# Autodesk Inventor assembly: RFO-Mounted
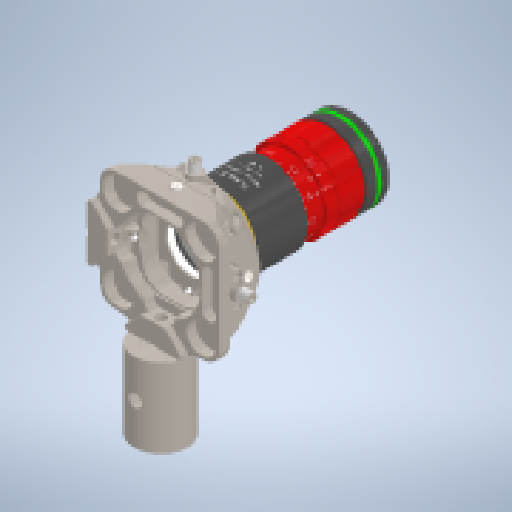
[picture p0: Inventor's stored thumbnail of the model, 512x512]
Saved by Autodesk Inventor 2024.2 (Build 282272000, 272)
## iProperties
Created: 2024-11-27
Part Number: RFO-Mounted
Document SubType Name: Assembly
Designer: monolithic
Author: monolithic
## Documents named in this file (5)
- C:\Users\monolithic\Documents\GitHub\CAD\Monolith\John\ASLM_SampleScanning_Baseplate\Assembly\Components\SubAssemblies\RFO-Mounted.iam
- C:\Users\monolithic\Documents\GitHub\CAD\Monolith\John\ASLM_SampleScanning_Baseplate\Assembly\Components\SubAssemblies\PLS-P150.ipt
- C:\Users\monolithic\Documents\GitHub\CAD\Monolith\John\ASLM_SampleScanning_Baseplate\Assembly\Components\SubAssemblies\POLARIS-1XY.ipt
- C:\Users\monolithic\Documents\GitHub\CAD\Monolith\John\ASLM_SampleScanning_Baseplate\Assembly\Components\SubAssemblies\TL15X-2P-Step.ipt
- C:\Users\monolithic\Documents\GitHub\CAD\Monolith\John\ASLM_SampleScanning_Baseplate\Assembly\Components\SubAssemblies\SM1A34-Step.ipt
## Components (4 placed, 4 different names)
1. PLS-P150:1 — Mate:1, Mate:2
2. POLARIS-1XY:1 — Mate:1, Mate:2, Mate:3, Mate:4, Mate:6
3. TL15X-2P-Step:1 — Mate:5, Mate:6
4. SM1A34-Step:1 — Mate:3, Mate:4, Mate:5
## Relationships (6: Mate 6)
- Mate:1: PLS-P150:1 ↔ POLARIS-1XY:1
- Mate:2: PLS-P150:1 ↔ POLARIS-1XY:1
- Mate:3: POLARIS-1XY:1 ↔ SM1A34-Step:1
- Mate:4: POLARIS-1XY:1 ↔ SM1A34-Step:1
- Mate:5: TL15X-2P-Step:1 ↔ SM1A34-Step:1
- Mate:6: POLARIS-1XY:1 ↔ TL15X-2P-Step:1
